# Autodesk Inventor assembly: hubjig
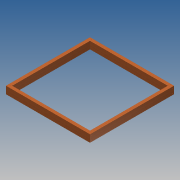
[picture p0: Inventor's stored thumbnail of the model, 180x180]
Saved by Autodesk Inventor 2014 SP1 (Build 180222100, 222)
## iProperties
Created: 2014-08-29
Part Number: hubjig
Document SubType Name: Assembly
Designer: Dave
Author: Dave
## Documents named in this file (3)
- C:\Users\Dave\Desktop\hera-cad\jigs\hubjig.iam
- C:\Users\Dave\Desktop\hera-cad\jigs\hubjig_side1.ipt
- C:\Users\Dave\Desktop\hera-cad\jigs\hubjig_side2.ipt
## Components (4 placed, 2 different names)
1. hubjig_side1:1 — Insert:1, Insert:2
2. hubjig_side2:1 — Insert:1, Insert:3
3. hubjig_side2:2 — Insert:2
4. hubjig_side1:2 — Insert:3
## Relationships (3: Insert 3)
- Insert:1: hubjig_side1:1 ↔ hubjig_side2:1
- Insert:2: hubjig_side1:1 ↔ hubjig_side2:2
- Insert:3: hubjig_side2:1 ↔ hubjig_side1:2
